# Autodesk Inventor assembly: Ramps + Arduino + Adapter
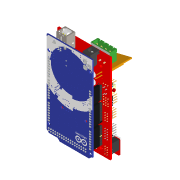
[picture p0: Inventor's stored thumbnail of the model, 180x180]
Saved by Autodesk Inventor 2020 (Build 240168000, 168)
## iProperties
Created: 2020-06-20
Part Number: Ramps + Arduino + Adapter
Document SubType Name: Assembly
Designer: Dante
Author: Dante
## Documents named in this file (4)
- C:\Users\Hernan\Documents\Ciclo Lectivo 2020 - I.I.L.A.H\Router CNC\Etapa 4\Diseños Autodesk Inventor\Ensambles\Ensamble Ajuste Fino Total + Elect. - Act. 29_9_2020\Componentes Electrónicos\Ramps + Arduino + Adapter.iam
- C:\Users\Hernan\Documents\Ciclo Lectivo 2020 - I.I.L.A.H\Router CNC\Etapa 4\Diseños Autodesk Inventor\Ensambles\Ensamble Ajuste Fino Total + Elect. - Act. 29_9_2020\Componentes Electrónicos\Arduino MEGA 2560 R3.ipt
- C:\Users\Hernan\Documents\Ciclo Lectivo 2020 - I.I.L.A.H\Router CNC\Etapa 4\Diseños Autodesk Inventor\Ensambles\Ensamble Ajuste Fino Total + Elect. - Act. 29_9_2020\Componentes Electrónicos\Shield Ramps 1.4.ipt
- C:\Users\Hernan\Documents\Ciclo Lectivo 2020 - I.I.L.A.H\Router CNC\Etapa 4\Diseños Autodesk Inventor\Ensambles\Ensamble Ajuste Fino Total + Elect. - Act. 29_9_2020\Componentes Electrónicos\Smart adapter conector LCD Ramps 1.4.ipt
## Components (3 placed, 3 different names)
1. Arduino MEGA 2560 R3:1 — Mate:1, Flush:1, Mate:2
2. Shield Ramps 1.4:1 — Mate:1, Flush:1, Mate:2, Mate:3, Mate:4, Flush:2
3. Smart adapter conector LCD Ramps 1.4:1 — Mate:3, Mate:4, Flush:2
## Relationships (6: Mate 4, Flush 2)
- Mate:1: Arduino MEGA 2560 R3:1 ↔ Shield Ramps 1.4:1
- Flush:1: Arduino MEGA 2560 R3:1 ↔ Shield Ramps 1.4:1
- Mate:2: Arduino MEGA 2560 R3:1 ↔ Shield Ramps 1.4:1
- Mate:3: Shield Ramps 1.4:1 ↔ Smart adapter conector LCD Ramps 1.4:1
- Mate:4: Shield Ramps 1.4:1 ↔ Smart adapter conector LCD Ramps 1.4:1
- Flush:2: Shield Ramps 1.4:1 ↔ Smart adapter conector LCD Ramps 1.4:1
